# Autodesk Inventor assembly: Assembly444
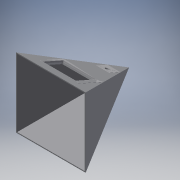
[picture p0: Inventor's stored thumbnail of the model, 180x180]
Saved by Autodesk Inventor 2018 (Build 220112000, 112)
## iProperties
Created: 2019-03-15
Part Number: Assembly444
Document SubType Name: Assembly
Designer: hryst
Author: hryst
## Documents named in this file (4)
- C:\Users\hryst\Google Drive\Me\AI\GestureRecognition\3D_pyramid\Assembly444.iam
- C:\Users\hryst\Google Drive\Me\AI\GestureRecognition\3D_pyramid\pyramid.ipt
- C:\Users\hryst\Google Drive\Me\AI\GestureRecognition\3D_pyramid\raspi_case_top.ipt
- C:\Users\hryst\Google Drive\Me\AI\GestureRecognition\3D_pyramid\camera_case_front_inv.ipt
## Components (3 placed, 3 different names)
1. pyramid:1 — Flush:1, Flush:2, Flush:3
2. raspi_case_top:1 — Flush:1, Flush:2
3. camera_case_front_inv:1 — Flush:3
## Relationships (3: Flush 3)
- Flush:1: pyramid:1 ↔ raspi_case_top:1
- Flush:2: pyramid:1 ↔ raspi_case_top:1
- Flush:3: pyramid:1 ↔ camera_case_front_inv:1
